# Autodesk Inventor assembly: remote button
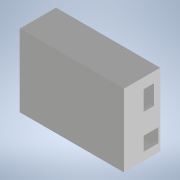
[picture p0: Inventor's stored thumbnail of the model, 180x180]
Saved by Autodesk Inventor 2021 (Build 250183000, 183)
## iProperties
Created: 2021-10-26
Part Number: remote button
Document SubType Name: Assembly
Designer: eddys
Author: eddys
## Documents named in this file (3)
- C:\Users\eddys\Desktop\remote switch\remote button.iam
- C:\Users\eddys\Desktop\remote switch\remotebuttonbox.ipt
- C:\Users\eddys\Desktop\remote switch\remotebuttonlid.ipt
## Components (2 placed, 2 different names)
1. remotebuttonbox:1 — Mate:1, Flush:1, Flush:2
2. remotebuttonlid:1 — Mate:1, Flush:1, Flush:2
## Relationships (3: Flush 2, Mate 1)
- Mate:1: remotebuttonbox:1 ↔ remotebuttonlid:1
- Flush:1: remotebuttonbox:1 ↔ remotebuttonlid:1
- Flush:2: remotebuttonbox:1 ↔ remotebuttonlid:1
